# Autodesk Inventor assembly: Fan Assembly
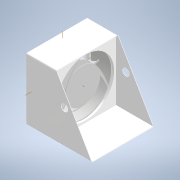
[picture p0: Inventor's stored thumbnail of the model, 180x180]
Saved by Autodesk Inventor 2021 (Build 250183000, 183)
## iProperties
Created: 2020-12-03
Part Number: Fan Assembly
Document SubType Name: Assembly
Designer: leoulgezu18
Author: leoulgezu18
## Documents named in this file (3)
- C:\Users\leoul\Desktop\Kinect 3D Modeling-20201204T005715Z-001\Kinect 3D Modeling\Sub-assemblies\Fan Assembly.iam
- C:\Users\leoul\Desktop\Kinect 3D Modeling-20201204T005715Z-001\Kinect 3D Modeling\Parts\Fan Inner.ipt
- C:\Users\leoul\Desktop\Kinect 3D Modeling-20201204T005715Z-001\Kinect 3D Modeling\Parts\Fan Outer.ipt
## Components (2 placed, 2 different names)
1. Fan Inner:1 — Angle:1, Flush:1, Mate:1
2. Fan Outer:1 — Angle:1, Flush:1, Mate:1
## Relationships (3: Angle 1, Flush 1, Mate 1)
- Angle:1 (0 deg): Fan Inner:1 ↔ Fan Outer:1
- Flush:1 (2.54 mm): Fan Inner:1 ↔ Fan Outer:1
- Mate:1: Fan Inner:1 ↔ Fan Outer:1
